# Autodesk Inventor assembly: AssemblyV3
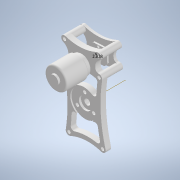
[picture p0: Inventor's stored thumbnail of the model, 180x180]
Saved by Autodesk Inventor 2022 (Build 260153070, 153G)
## iProperties
Created: 2021-11-03
Part Number: AssemblyV3
Document SubType Name: Assembly
Designer: a laptop
Author: a laptop
## Documents named in this file (12)
- C:\Users\a laptop\Desktop\SumoBot\sumobotLIDAR\AssemblyV3.iam
- C:\Users\a laptop\Desktop\SumoBot\sumobotLIDAR\AssemblyV3\Design Accelerator\Spur Gears1.iam
- C:\Users\a laptop\Desktop\SumoBot\sumobotLIDAR\BigGear54T.ipt
- C:\Users\a laptop\Desktop\SumoBot\sumobotLIDAR\SmallGear9T.ipt
- C:\Users\a laptop\Desktop\SumoBot\sumobotLIDAR\REF_PART\VL53L1X board.ipt
- C:\Users\a laptop\Desktop\SumoBot\sumobotLIDAR\REF_PART\Magnet.ipt
- C:\Users\a laptop\Desktop\SumoBot\sumobotLIDAR\REF_PART\AS5600.ipt
- C:\Users\a laptop\Desktop\SumoBot\sumobotLIDAR\AS5600_mount.ipt
- C:\Users\a laptop\Desktop\SumoBot\sumobotLIDAR\REF_PART\608ZZ bearing.ipt
- C:\Users\a laptop\Desktop\SumoBot\sumobotLIDAR\AdapterLplateV2.ipt
- C:\Users\a laptop\Desktop\SumoBot\sumobotLIDAR\REF_PART\MOTOR.ipt
- C:\Users\a laptop\Desktop\SumoBot\sumobotLIDAR\REF_PART\SRM-12-06A.ipt
## Components (11 placed, 11 different names)
1. Spur Gears:1 [sub-assembly]
2. BigGear54T:1 — Mate:1, Rotation:1, Mate:3, Angle:2, Flush:1, Angle:3, Flush:2, Mate:4, Mate:5, Mate:14
3. SmallGear9T:1 — Mate:1, Rotation:1, Mate:2, Angle:1, Flush:1, Mate:6, Mate:7, Mate:15, Mate:16
4. VL53L1X board:1 — Angle:3, Flush:2, Mate:4, Mate:5
5. Magnet:1 — Mate:6, Mate:7, Mate:8, Mate:9
6. AS5600:1 — Mate:8, Mate:9, Mate:26, Mate:27, Mate:28, Mate:29
7. AS5600_mount:1 — Mate:27, Mate:28, Mate:29
8. 608ZZ bearing:1 — Mate:13, Mate:14
9. MOTOR:1 — Mate:15, Mate:16, Mate:22
10. SRM-12-06A:1 — Mate:22, Flush:3, Mate:23, Mate:30
11. AdapterLplateV2:1 — Flush:3, Mate:23
## Relationships (32: Mate 24, Angle 4, Flush 3, RelateRotation 1)
- Mate:1 (32.308 mm): BigGear54T:1 ↔ SmallGear9T:1
- Rotation:1 [RelateRotation] (6 ul): BigGear54T:1 ↔ SmallGear9T:1
- Mate:2: SmallGear9T:1
- Angle:1 (0 deg): SmallGear9T:1
- Mate:3: BigGear54T:1
- Angle:2 (0 deg): BigGear54T:1
- Flush:1: BigGear54T:1 ↔ SmallGear9T:1
- Angle:3 (0 deg): BigGear54T:1 ↔ VL53L1X board:1
- Flush:2: BigGear54T:1 ↔ VL53L1X board:1
- Mate:4: BigGear54T:1 ↔ VL53L1X board:1
- Mate:5 (-35 mm): BigGear54T:1 ↔ VL53L1X board:1
- Mate:6: SmallGear9T:1 ↔ Magnet:1
- Mate:7: SmallGear9T:1 ↔ Magnet:1
- Mate:8: Magnet:1 ↔ AS5600:1
- Mate:9 (0.5 mm): Magnet:1 ↔ AS5600:1
- Mate:13: 608ZZ bearing:1
- Mate:14: BigGear54T:1 ↔ 608ZZ bearing:1
- Mate:15 (1 mm): SmallGear9T:1 ↔ MOTOR:1
- Mate:16: SmallGear9T:1 ↔ MOTOR:1
- Mate:20
- Mate:21
- Angle:5 (0 deg)
- Mate:22: MOTOR:1 ↔ SRM-12-06A:1
- Flush:3: SRM-12-06A:1 ↔ AdapterLplateV2:1
- Mate:23: SRM-12-06A:1 ↔ AdapterLplateV2:1
- Mate:24
- Mate:25
- Mate:26: AS5600:1
- Mate:27: AS5600:1 ↔ AS5600_mount:1
- Mate:28: AS5600:1 ↔ AS5600_mount:1
- Mate:29: AS5600:1 ↔ AS5600_mount:1
- Mate:30: SRM-12-06A:1
